# Autodesk Inventor assembly: mechanical assembly
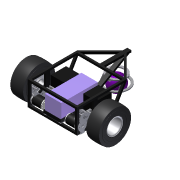
[picture p0: Inventor's stored thumbnail of the model, 180x180]
Saved by Autodesk Inventor 2012 (Build 160160000, 160)
## iProperties
Created: 2011-09-30
Part Number: mechanical assembly
Document SubType Name: Assembly
Designer: Antonella
Author: Antonella
## Documents named in this file (13)
- C:\Users\Antonella\Documents\GCC Robotics 2012 - Mechanical\Robot 2.0\mechanical assembly.iam
- C:\Users\Antonella\Documents\GCC Robotics 2012 - Mechanical\Robot 2.0\Chassis\chassis weldment.iam
- C:\Users\Antonella\Documents\GCC Robotics 2012 - Mechanical\Robot 2.0\Drive Train\Turf Tire\wheel kenda turf tire.iam
- C:\Users\Antonella\Documents\GCC Robotics 2012 - Mechanical\Robot 2.0\Payload Mount\payload mount.iam
- C:\Users\Antonella\Documents\GCC Robotics 2012 - Mechanical\Robot 2.0\Drive Train\Gearbox\gearbox.iam
- C:\Users\Antonella\Documents\GCC Robotics 2012 - Mechanical\Robot 2.0\Electrical\battery model.ipt
- C:\Users\Antonella\Documents\GCC Robotics 2012 - Mechanical\Robot 2.0\Drive Train\bearing block wheel mount.iam
- C:\Users\Antonella\Documents\GCC Robotics 2012 - Mechanical\Robot 2.0\Drive Train\Gearbox\gearbox_MIR.iam
- C:\Users\Antonella\Documents\GCC Robotics 2012 - Mechanical\Robot 2.0\Ball Caster\ball caster.iam
- C:\Users\Antonella\Documents\GCC Robotics 2012 - Mechanical\Robot 2.0\Drive Train\wheel_shaft.ipt
- C:\Users\Antonella\Documents\GCC Robotics 2012 - Mechanical\Robot 2.0\Drive Train\wheel_hub.ipt
- C:\Users\Antonella\Documents\GCC Robotics 2012 - Mechanical\Robot 2.0\Drive Train\sprocket_rollerchain_30t x 25p.ipt
- C:\Users\Antonella\Documents\GCC Robotics 2012 - Mechanical\Robot 2.0\Drive Train\bearing block wheel mount inner.iam
## Components (19 placed, 12 different names)
1. chassis weldment:1 [sub-assembly] — Mate:20, Flush:6, Mate:21, Flush:7, Mate:39, Flush:9, Mate:40, Mate:43, Mate:44, Mate:45, Mate:46, Mate:47, Mate:48, Mate:49, Mate:50, Mate:51, Mate:52, Mate:53, Mate:54, Mate:55, Flush:11, Mate:56, Mate:57, Mate:58, Mate:71, Angle:1, Mate:73, Mate:74, Angle:2
2. wheel kenda turf tire:1 [sub-assembly] — Mate:75, Mate:76
3. wheel kenda turf tire:2 [sub-assembly] — Mate:69, Mate:70
4. payload mount:1 [sub-assembly] — Mate:20, Flush:6, Mate:21, Flush:7
5. gearbox:1 [sub-assembly] — Mate:49, Mate:50, Mate:51, Flush:14
6. gearbox_MIR:1 [sub-assembly] — Mate:52, Mate:53, Mate:54, Flush:15
7. ball caster:1 [sub-assembly] — Mate:57, Mate:58
8. battery model:1 — Mate:39, Flush:9, Mate:40
9. battery model:2 — Mate:55, Flush:11, Mate:56
10. bearing block wheel mount:1 [sub-assembly] — Mate:43, Mate:44, Mate:45, Mate:67
11. bearing block wheel mount:2 [sub-assembly] — Mate:46, Mate:47, Mate:48, Mate:59
12. wheel_shaft:1 — Mate:59, Mate:60, Flush:12, Mate:61
13. wheel_shaft:2 — Mate:67, Flush:13, Mate:68, Mate:72
14. wheel_hub:1 — Mate:60, Flush:12, Mate:62, Mate:63, Mate:75, Mate:76
15. wheel_hub:2 — Mate:64, Mate:65, Mate:66, Flush:13, Mate:68, Mate:69, Mate:70
16. Roller Chain Sprocket2:1 — Mate:64, Mate:65, Mate:66, Flush:14
17. Roller Chain Sprocket2:2 — Mate:61, Mate:62, Mate:63, Flush:15
18. bearing block wheel mount inner:1 [sub-assembly] — Mate:73, Mate:74, Angle:2
19. bearing block wheel mount inner:2 [sub-assembly] — Mate:71, Mate:72, Angle:1
## Relationships (48: Mate 38, Flush 8, Angle 2)
- Mate:20: chassis weldment:1 ↔ payload mount:1
- Flush:6: chassis weldment:1 ↔ payload mount:1
- Mate:21: chassis weldment:1 ↔ payload mount:1
- Flush:7: chassis weldment:1 ↔ payload mount:1
- Mate:39: chassis weldment:1 ↔ battery model:1
- Flush:9: chassis weldment:1 ↔ battery model:1
- Mate:40: chassis weldment:1 ↔ battery model:1
- Mate:43: chassis weldment:1 ↔ bearing block wheel mount:1
- Mate:44: chassis weldment:1 ↔ bearing block wheel mount:1
- Mate:45: chassis weldment:1 ↔ bearing block wheel mount:1
- Mate:46: chassis weldment:1 ↔ bearing block wheel mount:2
- Mate:47: chassis weldment:1 ↔ bearing block wheel mount:2
- Mate:48: chassis weldment:1 ↔ bearing block wheel mount:2
- Mate:49: chassis weldment:1 ↔ gearbox:1
- Mate:50: chassis weldment:1 ↔ gearbox:1
- Mate:51: chassis weldment:1 ↔ gearbox:1
- Mate:52: chassis weldment:1 ↔ gearbox_MIR:1
- Mate:53: chassis weldment:1 ↔ gearbox_MIR:1
- Mate:54: chassis weldment:1 ↔ gearbox_MIR:1
- Mate:55: chassis weldment:1 ↔ battery model:2
- Flush:11: chassis weldment:1 ↔ battery model:2
- Mate:56: chassis weldment:1 ↔ battery model:2
- Mate:57: chassis weldment:1 ↔ ball caster:1
- Mate:58 (-25.4 mm): chassis weldment:1 ↔ ball caster:1
- Mate:59: bearing block wheel mount:2 ↔ wheel_shaft:1
- Mate:60: wheel_shaft:1 ↔ wheel_hub:1
- Flush:12: wheel_shaft:1 ↔ wheel_hub:1
- Mate:61: wheel_shaft:1 ↔ Roller Chain Sprocket2:2
- Mate:62: wheel_hub:1 ↔ Roller Chain Sprocket2:2
- Mate:63: wheel_hub:1 ↔ Roller Chain Sprocket2:2
- Mate:64: wheel_hub:2 ↔ Roller Chain Sprocket2:1
- Mate:65: wheel_hub:2 ↔ Roller Chain Sprocket2:1
- Mate:66: wheel_hub:2 ↔ Roller Chain Sprocket2:1
- Mate:67: bearing block wheel mount:1 ↔ wheel_shaft:2
- Flush:13: wheel_shaft:2 ↔ wheel_hub:2
- Mate:68: wheel_shaft:2 ↔ wheel_hub:2
- Mate:69: wheel kenda turf tire:2 ↔ wheel_hub:2
- Mate:70: wheel kenda turf tire:2 ↔ wheel_hub:2
- Mate:71: chassis weldment:1 ↔ bearing block wheel mount inner:2
- Mate:72: wheel_shaft:2 ↔ bearing block wheel mount inner:2
- Angle:1 (0 deg): chassis weldment:1 ↔ bearing block wheel mount inner:2
- Mate:73: chassis weldment:1 ↔ bearing block wheel mount inner:1
- Mate:74: chassis weldment:1 ↔ bearing block wheel mount inner:1
- Angle:2 (0 deg): chassis weldment:1 ↔ bearing block wheel mount inner:1
- Flush:14: gearbox:1 ↔ Roller Chain Sprocket2:1
- Mate:75: wheel kenda turf tire:1 ↔ wheel_hub:1
- Mate:76: wheel kenda turf tire:1 ↔ wheel_hub:1
- Flush:15: gearbox_MIR:1 ↔ Roller Chain Sprocket2:2
